# Autodesk Inventor assembly: GE-12100
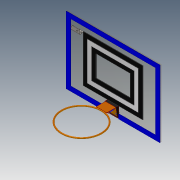
[picture p0: Inventor's stored thumbnail of the model, 180x180]
Saved by Autodesk Inventor 2012 (Build 160160000, 160)
## iProperties
Created: 2011-10-28
Part Number: GE-12100
Document SubType Name: Assembly
Designer: dfoster
Description: Backboard Assembly, Right
Title: Backboard Assembly, Right
Author: dfoster
## Documents named in this file (11)
- C:\Data Folder\FRC 2012 Field\Components\GE-12100.iam
- C:\Data Folder\FRC 2012 Field\Components\GE-12073.ipt
- C:\Data Folder\FRC 2012 Field\Components\GE-12013.ipt
- C:\Data Folder\FRC 2012 Field\Components\GE-12098-01.ipt
- C:\Data Folder\FRC 2012 Field\Components\GE-12098-02.ipt
- C:\Data Folder\FRC 2012 Field\Components\HW-00013.ipt
- C:\Data Folder\FRC 2012 Field\Components\HW-00002.ipt
- C:\Data Folder\FRC 2012 Field\Components\HW-00037.ipt
- C:\Data Folder\FRC 2012 Field\Components\HW-00033.ipt
- C:\Data Folder\FRC 2012 Field\Components\HW-00039.ipt
- C:\Data Folder\FRC 2012 Field\Components\GE-12074.ipt
## Components (30 placed, 10 different names)
1. GE-12074:1 — Mate:1, Mate:2, Mate:3, Mate:4, Mate:5, Mate:6, Mate:7, Mate:8, Mate:9, Mate:10, Flush:1, Flush:2, Mate:11, Flush:3, Mate:13, Flush:4, Flush:5, Insert:5
2. GE-12073:1 — Mate:4, Mate:6, Mate:7, Mate:14, Insert:2
3. GE-12073:2 — Mate:5, Mate:8, Mate:9, Insert:1
4. GE-12013:1 — Mate:1, Mate:2, Mate:3, Mate:12, Insert:3
5. GE-12098-01:1 — Mate:10, Flush:1, Flush:2
6. GE-12098-02:1 — Mate:11, Mate:12, Flush:3
7. HW-00013:1 — Mate:13, Flush:4
8. HW-00002:1 — Insert:1
9. HW-00013:2 — Flush:5, Mate:14
10. HW-00002:2 — Insert:2
11. HW-00013:3
12. HW-00002:3
13. HW-00013:4
14. HW-00002:4
15. HW-00037:1 — Insert:4
16. HW-00033:1 — Insert:6
17. HW-00039:1 — Insert:3, Insert:4
18. HW-00039:2 — Insert:5, Insert:6
19. HW-00037:2
20. HW-00033:2
21. HW-00039:3
22. HW-00039:4
23. HW-00037:3
24. HW-00033:3
25. HW-00039:5
26. HW-00039:6
27. HW-00037:4
28. HW-00033:4
29. HW-00039:7
30. HW-00039:8
## Component patterns: (2 elements, first: HW-00013:1 + HW-00002:1 + HW-00013:2 + HW-00002:2), (4 elements, first: HW-00037:1 + HW-00033:1 + HW-00039:1 + HW-00039:2)
## Relationships (25: Mate 14, Insert 6, Flush 5)
- Mate:1: GE-12074:1 ↔ GE-12013:1
- Mate:2: GE-12074:1 ↔ GE-12013:1
- Mate:3: GE-12074:1 ↔ GE-12013:1
- Mate:4: GE-12074:1 ↔ GE-12073:1
- Mate:5: GE-12074:1 ↔ GE-12073:2
- Mate:6: GE-12074:1 ↔ GE-12073:1
- Mate:7: GE-12074:1 ↔ GE-12073:1
- Mate:8: GE-12074:1 ↔ GE-12073:2
- Mate:9: GE-12074:1 ↔ GE-12073:2
- Mate:10: GE-12074:1 ↔ GE-12098-01:1
- Flush:1: GE-12074:1 ↔ GE-12098-01:1
- Flush:2: GE-12074:1 ↔ GE-12098-01:1
- Mate:11: GE-12074:1 ↔ GE-12098-02:1
- Mate:12: GE-12013:1 ↔ GE-12098-02:1
- Flush:3 (203.2 mm): GE-12074:1 ↔ GE-12098-02:1
- Mate:13: GE-12074:1 ↔ HW-00013:1
- Flush:4: GE-12074:1 ↔ HW-00013:1
- Insert:1: GE-12073:2 ↔ HW-00002:1
- Flush:5: GE-12074:1 ↔ HW-00013:2
- Mate:14: GE-12073:1 ↔ HW-00013:2
- Insert:2: GE-12073:1 ↔ HW-00002:2
- Insert:3: GE-12013:1 ↔ HW-00039:1
- Insert:4: HW-00037:1 ↔ HW-00039:1
- Insert:5: GE-12074:1 ↔ HW-00039:2
- Insert:6: HW-00033:1 ↔ HW-00039:2
